# Autodesk Inventor assembly: 4x2inTractionWheel.1111-2016
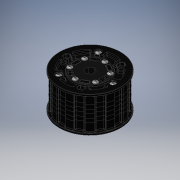
[picture p0: Inventor's stored thumbnail of the model, 180x180]
Saved by Autodesk Inventor 2016 SP1 (Build 200210100, 210)
## iProperties
Created: 2016-11-21
Part Number: 4x2inTractionWheel.1111-2016
Document SubType Name: Assembly
Designer: 589013
Author: 589013
## Documents named in this file (9)
- H:\PHRC\GrabCAD\VexproResources-1111-2016_17\_ORGANIZED AND LABELED FILES\Wheels\4 inch\4x2inTractionWheel.1111-2016.iam
- H:\PHRC\GrabCAD\VexproResources-1111-2016_17\_ORGANIZED AND LABELED FILES\Wheels\Wheel Parts\4InchWheelEnd.1111-2016.ipt
- H:\PHRC\GrabCAD\VexproResources-1111-2016_17\_ORGANIZED AND LABELED FILES\Fasteners\Screws\Screw8-32x1.25in.1111-2016.ipt
- H:\PHRC\GrabCAD\VexproResources-1111-2016_17\_ORGANIZED AND LABELED FILES\Fasteners\Nuts\Nut8-32Nylock.1111-2016.ipt
- H:\PHRC\GrabCAD\VexproResources-1111-2016_17\_ORGANIZED AND LABELED FILES\Versa Motion\VersaHub(0.5inHex)-1111-2016.ipt
- H:\PHRC\GrabCAD\VexproResources-1111-2016_17\_ORGANIZED AND LABELED FILES\Versa Motion\VersaHub(0.5inHex,Plastic)-1111-2016.ipt
- H:\PHRC\GrabCAD\VexproResources-1111-2016_17\_ORGANIZED AND LABELED FILES\Fasteners\Screws\Screw8-32x0.5in.1111-2016.ipt
- H:\PHRC\GrabCAD\VexproResources-1111-2016_17\_ORGANIZED AND LABELED FILES\Wheels\Wheel Parts\4InchWheelSpacer-1111-2016.ipt
- H:\PHRC\GrabCAD\VexproResources-1111-2016_17\_ORGANIZED AND LABELED FILES\Fasteners\Standoffs\Standoff1.75in(cut 2.00in)-1111-2016.ipt
## Components (30 placed, 8 different names)
1. 4InchWheelEnd.1111-2016:1 — Rotational:1, Angle:1, Rotational:4, Rotational:5, Rotational:6, Angle:2, Angle:3, Angle:4, Rotational:9, Rotational:10, Rotational:11, Rotational:12
2. 4InchWheelEnd.1111-2016:2 — Insert:1, Insert:2, Insert:3, Rotational:7, Rotational:8, Rotational:15, Rotational:16
3. Screw8-32x1.25in.1111-2016:1 — Insert:1
4. Screw8-32x1.25in.1111-2016:2 — Insert:2
5. Screw8-32x1.25in.1111-2016:3 — Insert:3
6. Nut8-32Nylock.1111-2016:1 — Rotational:6, Angle:2
7. Nut8-32Nylock.1111-2016:2 — Rotational:5, Angle:4
8. Nut8-32Nylock.1111-2016:3 — Rotational:4, Angle:3
9. VersaHub(0.5inHex)-1111-2016:1 — Rotational:7, Rotational:8, Insert:4, Insert:5, Insert:6, Insert:7, Insert:8, Insert:9
10. VersaHub(0.5inHex,Plastic)-1111-2016:1 — Rotational:9, Rotational:10, Insert:10, Insert:11, Insert:12, Insert:13, Insert:14, Insert:15
11. Screw8-32x0.5in.1111-2016:1 — Insert:4
12. Screw8-32x0.5in.1111-2016:2 — Insert:6
13. Screw8-32x0.5in.1111-2016:3 — Insert:5
14. Screw8-32x0.5in.1111-2016:4 — Insert:7
15. Screw8-32x0.5in.1111-2016:5 — Insert:8
16. Screw8-32x0.5in.1111-2016:6 — Insert:9
17. Screw8-32x0.5in.1111-2016:7 — Insert:10
18. Screw8-32x0.5in.1111-2016:8 — Insert:11
19. Screw8-32x0.5in.1111-2016:9 — Insert:13
20. Screw8-32x0.5in.1111-2016:10 — Insert:14
21. Screw8-32x0.5in.1111-2016:11 — Insert:12
22. Screw8-32x0.5in.1111-2016:12 — Insert:15
23. 4InchWheelSpacer-1111-2016:1 — Rotational:11, Rotational:12, Rotational:13, Rotational:14
24. 4InchWheelSpacer-1111-2016:2 — Rotational:13, Rotational:14, Rotational:15, Rotational:16
25. Standoff1.75in(cut 2.00in)-1111-2016:1 — Rotational:1, Angle:1
26. Standoff1.75in(cut 2.00in)-1111-2016:2
27. Standoff1.75in(cut 2.00in)-1111-2016:3
28. Standoff1.75in(cut 2.00in)-1111-2016:4
29. Standoff1.75in(cut 2.00in)-1111-2016:5
30. Standoff1.75in(cut 2.00in)-1111-2016:6
## Component patterns: (6 elements, first: Standoff1.75in(cut 2.00in)-1111-2016:1)
## Relationships (33: Insert 15, RevoluteJoint 14, Angle 4)
- Rotational:1 [RevoluteJoint]: 4InchWheelEnd.1111-2016:1 ↔ Standoff1.75in(cut 2.00in)-1111-2016:1
- Angle:1 (0 deg): 4InchWheelEnd.1111-2016:1 ↔ Standoff1.75in(cut 2.00in)-1111-2016:1
- Insert:1: 4InchWheelEnd.1111-2016:2 ↔ Screw8-32x1.25in.1111-2016:1
- Insert:2: 4InchWheelEnd.1111-2016:2 ↔ Screw8-32x1.25in.1111-2016:2
- Insert:3: 4InchWheelEnd.1111-2016:2 ↔ Screw8-32x1.25in.1111-2016:3
- Rotational:4 [RevoluteJoint]: 4InchWheelEnd.1111-2016:1 ↔ Nut8-32Nylock.1111-2016:3
- Rotational:5 [RevoluteJoint]: 4InchWheelEnd.1111-2016:1 ↔ Nut8-32Nylock.1111-2016:2
- Rotational:6 [RevoluteJoint]: 4InchWheelEnd.1111-2016:1 ↔ Nut8-32Nylock.1111-2016:1
- Angle:2 (0 deg): 4InchWheelEnd.1111-2016:1 ↔ Nut8-32Nylock.1111-2016:1
- Angle:3 (0 deg): 4InchWheelEnd.1111-2016:1 ↔ Nut8-32Nylock.1111-2016:3
- Angle:4 (0 deg): 4InchWheelEnd.1111-2016:1 ↔ Nut8-32Nylock.1111-2016:2
- Rotational:7 [RevoluteJoint]: 4InchWheelEnd.1111-2016:2 ↔ VersaHub(0.5inHex)-1111-2016:1
- Rotational:8 [RevoluteJoint]: 4InchWheelEnd.1111-2016:2 ↔ VersaHub(0.5inHex)-1111-2016:1
- Rotational:9 [RevoluteJoint]: 4InchWheelEnd.1111-2016:1 ↔ VersaHub(0.5inHex,Plastic)-1111-2016:1
- Rotational:10 [RevoluteJoint]: 4InchWheelEnd.1111-2016:1 ↔ VersaHub(0.5inHex,Plastic)-1111-2016:1
- Insert:4: VersaHub(0.5inHex)-1111-2016:1 ↔ Screw8-32x0.5in.1111-2016:1
- Insert:5: VersaHub(0.5inHex)-1111-2016:1 ↔ Screw8-32x0.5in.1111-2016:3
- Insert:6: VersaHub(0.5inHex)-1111-2016:1 ↔ Screw8-32x0.5in.1111-2016:2
- Insert:7: VersaHub(0.5inHex)-1111-2016:1 ↔ Screw8-32x0.5in.1111-2016:4
- Insert:8: VersaHub(0.5inHex)-1111-2016:1 ↔ Screw8-32x0.5in.1111-2016:5
- Insert:9: VersaHub(0.5inHex)-1111-2016:1 ↔ Screw8-32x0.5in.1111-2016:6
- Insert:10: VersaHub(0.5inHex,Plastic)-1111-2016:1 ↔ Screw8-32x0.5in.1111-2016:7
- Insert:11: VersaHub(0.5inHex,Plastic)-1111-2016:1 ↔ Screw8-32x0.5in.1111-2016:8
- Insert:12: VersaHub(0.5inHex,Plastic)-1111-2016:1 ↔ Screw8-32x0.5in.1111-2016:11
- Insert:13: VersaHub(0.5inHex,Plastic)-1111-2016:1 ↔ Screw8-32x0.5in.1111-2016:9
- Insert:14: VersaHub(0.5inHex,Plastic)-1111-2016:1 ↔ Screw8-32x0.5in.1111-2016:10
- Insert:15: VersaHub(0.5inHex,Plastic)-1111-2016:1 ↔ Screw8-32x0.5in.1111-2016:12
- Rotational:11 [RevoluteJoint]: 4InchWheelEnd.1111-2016:1 ↔ 4InchWheelSpacer-1111-2016:1
- Rotational:12 [RevoluteJoint]: 4InchWheelEnd.1111-2016:1 ↔ 4InchWheelSpacer-1111-2016:1
- Rotational:13 [RevoluteJoint]: 4InchWheelSpacer-1111-2016:1 ↔ 4InchWheelSpacer-1111-2016:2
- Rotational:14 [RevoluteJoint]: 4InchWheelSpacer-1111-2016:1 ↔ 4InchWheelSpacer-1111-2016:2
- Rotational:15 [RevoluteJoint]: 4InchWheelEnd.1111-2016:2 ↔ 4InchWheelSpacer-1111-2016:2
- Rotational:16 [RevoluteJoint]: 4InchWheelEnd.1111-2016:2 ↔ 4InchWheelSpacer-1111-2016:2
